# Autodesk Inventor assembly: ASY MSC 300.1 RIGHT BOARD
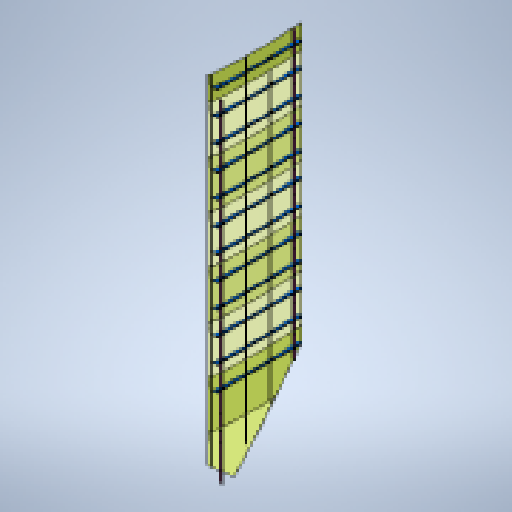
[picture p0: Inventor's stored thumbnail of the model, 512x512]
Saved by Autodesk Inventor 2025 (Build 290162010, 162A)
## iProperties
Created: 2024-07-22
Part Number: ASY MSC 300.1 RIGHT BOARD
Document SubType Name: Assembly
Designer: pokla
Stock Number: ASY МОО 300.1 правый борт
Mass: 330127 g
Surface Area: 285167 cm^2
Volume: 41265.8 cm^3
Density: 8 g/cm^3
Author: pokla
## Documents named in this file (10)
- C:\Users\admin\YandexDisk-badmisterfox\домашниий пк\Inventor\Manturovo\Manturovo_Se-clar\ASY MSC 203 RIGHT BOARD.iam
- C:\Users\admin\YandexDisk-badmisterfox\домашниий пк\Inventor\Manturovo\Manturovo_Se-clar\MSC 052 rib board.ipt
- C:\Users\admin\YandexDisk-badmisterfox\домашниий пк\Inventor\Manturovo\Manturovo_Se-clar\MSC 024 sheet board main.ipt
- C:\Users\admin\YandexDisk-badmisterfox\домашниий пк\Inventor\Manturovo\Manturovo_Se-clar\MSC 023 sheet board.ipt
- C:\Users\admin\YandexDisk-badmisterfox\домашниий пк\Inventor\Manturovo\Manturovo_Se-clar\MSC 025.2 sheet board withers.ipt
- C:\Users\admin\YandexDisk-badmisterfox\домашниий пк\Inventor\Manturovo\Manturovo_Se-clar\MSC 306 stringer BOARD  #.ipt
- C:\Users\admin\YandexDisk-badmisterfox\домашниий пк\Inventor\Manturovo\Manturovo_Se-clar\MSC 307 stringer BOARD  ##.ipt
- C:\Users\admin\YandexDisk-badmisterfox\домашниий пк\Inventor\Manturovo\Manturovo_Se-clar\MSC 027.2 sheet board withers 4.ipt
- C:\Users\admin\YandexDisk-badmisterfox\домашниий пк\Inventor\Manturovo\Manturovo_Se-clar\MSC 308 stringer BOARD  ###.ipt
- C:\Users\admin\YandexDisk-badmisterfox\домашниий пк\Inventor\Manturovo\Manturovo_Se-clar\MSC 309 stringer BOARD  ####.ipt
## Components (46 placed, 14 different names)
1. MSC 023 sheet board.ipt:1 — Flush:2, Flush:3, Flush:4, Rigid:1, Tangent:1, Mate:1
2. MSC 024 sheet board main.ipt:1 — Rigid:1, Rigid:2, Flush:5
3. MSC 024 sheet board main.ipt:2 — Rigid:2, Rigid:3
4. MSC 024 sheet board main.ipt:3 — Rigid:3, Rigid:4
5. MSC 024 sheet board main.ipt:4 — Rigid:4, Rigid:5
6. MSC 024 sheet board main.ipt:5 — Rigid:5, Rigid:19
7. MSC 025.2 sheet board withers.ipt:1 — Rigid:19, Rigid:20
8. MSC 027.2 sheet board withers 4.ipt:1 — Rigid:20
9. MSC 052 rib board.ipt:1 — Rigid:18, Tangent:1, Mate:1
10. MSC 052 rib board.ipt:2 — Rigid:12, Rigid:15, Rigid:16, Rigid:17
11. MSC 052 rib board.ipt:3 — Rigid:13
12. MSC 306 stringer BOARD  #.ipt:1 — Rigid:6, Rigid:12, Rigid:18
13. MSC 307 stringer BOARD  ##.ipt:1 — Rigid:7, Rigid:16, Flush:5
14. MSC 308 stringer BOARD  ###.ipt:1 — Rigid:8, Rigid:9
15. MSC 309 stringer BOARD  ####.ipt:1 — Rigid:10, Rigid:11
16. MSC 309 stringer BOARD  ####.ipt:2 — Rigid:10, Rigid:15
17. MSC 308 stringer BOARD  ###.ipt:2 — Rigid:8, Rigid:17
18. MSC 052 rib board.ipt:4 — Rigid:14
19. MSC 052 rib board:6
20. MSC 052 rib board:7
21. MSC 052 rib board:8
22. MSC 052 rib board:9
23. MSC 052 rib board:10
24. MSC 052 rib board:11
25. MSC 052 rib board:12
26. MSC 052 rib board:13
27. MSC 306 stringer BOARD  #.ipt:2 — Rigid:6, Rigid:13, Rigid:14
28. MSC 307 stringer BOARD  ##.ipt:2 — Rigid:7
29. MSC 308 stringer BOARD  ###.ipt:3 — Rigid:9
30. MSC 309 stringer BOARD  ####.ipt:3 — Rigid:11
31. MSC 306 stringer BOARD  #:3
32. MSC 307 stringer BOARD  ##:3
33. MSC 308 stringer BOARD  ###:4
34. MSC 309 stringer BOARD  ####:4
35. MSC 306 stringer BOARD  #:4
36. MSC 307 stringer BOARD  ##:4
37. MSC 308 stringer BOARD  ###:5
38. MSC 309 stringer BOARD  ####:5
39. MSC 306 stringer BOARD  #:5
40. MSC 307 stringer BOARD  ##:5
41. MSC 308 stringer BOARD  ###:6
42. MSC 309 stringer BOARD  ####:6
43. MSC 306 stringer BOARD  #:6
44. MSC 307 stringer BOARD  ##:6
45. MSC 308 stringer BOARD  ###:7
46. MSC 309 stringer BOARD  ####:7
## Component patterns: (9 elements, first: MSC 052 rib board.ipt:4), (5 elements, first: MSC 306 stringer BOARD  #.ipt:2 + MSC 307 stringer BOARD  ##.ipt:2 + MSC 308 stringer BOARD  ###.ipt:3 + MSC 309 stringer BOARD  ####.ipt:3)
## Relationships (26: WeldJoint 20, Flush 4, Tangent 1, Mate 1)
- Flush:2: MSC 023 sheet board.ipt:1
- Flush:3: MSC 023 sheet board.ipt:1
- Flush:4: MSC 023 sheet board.ipt:1
- Rigid:1 [WeldJoint]: MSC 023 sheet board.ipt:1 ↔ MSC 024 sheet board main.ipt:1
- Rigid:2 [WeldJoint]: MSC 024 sheet board main.ipt:1 ↔ MSC 024 sheet board main.ipt:2
- Rigid:3 [WeldJoint]: MSC 024 sheet board main.ipt:2 ↔ MSC 024 sheet board main.ipt:3
- Rigid:4 [WeldJoint]: MSC 024 sheet board main.ipt:3 ↔ MSC 024 sheet board main.ipt:4
- Rigid:5 [WeldJoint]: MSC 024 sheet board main.ipt:4 ↔ MSC 024 sheet board main.ipt:5
- Rigid:6 [WeldJoint]: MSC 306 stringer BOARD  #.ipt:1 ↔ MSC 306 stringer BOARD  #.ipt:2
- Rigid:7 [WeldJoint]: MSC 307 stringer BOARD  ##.ipt:1 ↔ MSC 307 stringer BOARD  ##.ipt:2
- Rigid:8 [WeldJoint]: MSC 308 stringer BOARD  ###.ipt:1 ↔ MSC 308 stringer BOARD  ###.ipt:2
- Rigid:9 [WeldJoint]: MSC 308 stringer BOARD  ###.ipt:1 ↔ MSC 308 stringer BOARD  ###.ipt:3
- Rigid:10 [WeldJoint]: MSC 309 stringer BOARD  ####.ipt:1 ↔ MSC 309 stringer BOARD  ####.ipt:2
- Rigid:11 [WeldJoint]: MSC 309 stringer BOARD  ####.ipt:1 ↔ MSC 309 stringer BOARD  ####.ipt:3
- Rigid:12 [WeldJoint] (2 mm): MSC 052 rib board.ipt:2 ↔ MSC 306 stringer BOARD  #.ipt:1
- Rigid:13 [WeldJoint] (2 mm): MSC 052 rib board.ipt:3 ↔ MSC 306 stringer BOARD  #.ipt:2
- Rigid:14 [WeldJoint] (2 mm): MSC 052 rib board.ipt:4 ↔ MSC 306 stringer BOARD  #.ipt:2
- Rigid:15 [WeldJoint] (2 mm): MSC 052 rib board.ipt:2 ↔ MSC 309 stringer BOARD  ####.ipt:2
- Rigid:16 [WeldJoint] (2 mm): MSC 052 rib board.ipt:2 ↔ MSC 307 stringer BOARD  ##.ipt:1
- Rigid:17 [WeldJoint] (2 mm): MSC 052 rib board.ipt:2 ↔ MSC 308 stringer BOARD  ###.ipt:2
- Rigid:18 [WeldJoint] (2 mm): MSC 052 rib board.ipt:1 ↔ MSC 306 stringer BOARD  #.ipt:1
- Rigid:19 [WeldJoint]: MSC 024 sheet board main.ipt:5 ↔ MSC 025.2 sheet board withers.ipt:1
- Rigid:20 [WeldJoint]: MSC 025.2 sheet board withers.ipt:1 ↔ MSC 027.2 sheet board withers 4.ipt:1
- Flush:5: MSC 024 sheet board main.ipt:1 ↔ MSC 307 stringer BOARD  ##.ipt:1
- Tangent:1: MSC 023 sheet board.ipt:1 ↔ MSC 052 rib board.ipt:1
- Mate:1 (75 mm): MSC 023 sheet board.ipt:1 ↔ MSC 052 rib board.ipt:1
